# Autodesk Inventor assembly: ArmAssembly
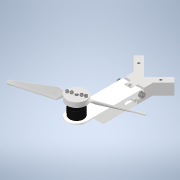
[picture p0: Inventor's stored thumbnail of the model, 180x180]
Saved by Autodesk Inventor 2021 (Build 250183000, 183)
## iProperties
Created: 2020-11-19
Part Number: ArmAssembly
Document SubType Name: Assembly
Designer: Pysion
Author: Pysion
## Documents named in this file (10)
- C:\Users\vineeth\Desktop\GrabCAD\Group 32 Assembly\ArmAssembly.iam
- C:\Users\vineeth\Desktop\GrabCAD\Group 32 Assembly\PropellerAssembly.iam
- C:\Users\vineeth\Desktop\GrabCAD\Group 32 Assembly\Motor.ipt
- C:\Users\vineeth\Desktop\GrabCAD\Group 32 Assembly\l_bracket.ipt
- C:\Users\vineeth\Desktop\GrabCAD\Group 32 Assembly\Motor Full Arm.ipt
- C:\Users\vineeth\Desktop\GrabCAD\Group 32 Assembly\slider.ipt
- C:\Users\vineeth\Desktop\GrabCAD\Group 32 Assembly\Compress Spring11.ipt
- C:\Users\vineeth\Desktop\GrabCAD\Group 32 Assembly\Pin GB 878-86 6 x 20.ipt
- C:\Users\vineeth\Desktop\GrabCAD\Group 32 Assembly\ContentCenter\en-US\AS 1420\AS 1420 - 1973 - M6 x 16.ipt
- C:\Users\vineeth\Documents\Inventor\Content Center Files\R2021\en-US\AS 1420\AS 1420 - 1973 - M4 x 10.ipt
## Components (14 placed, 9 different names)
1. PropellerAssembly:1 [sub-assembly] — Insert:1
2. Motor:1 — Mate:4, Mate:5, Mate:6, Insert:1
3. l_bracket:1 — Angle:1, Mate:8, Mate:21, Angle:3
4. Motor Full Arm:1 — Angle:1, Mate:4, Mate:5, Mate:6, Mate:8, Mate:17, Mate:18, Mate:19, Mate:20, Mate:21, Mate:22, Mate:23, Mate:24, Mate:25, Insert:2, Insert:3, Insert:4, Insert:5, Angle:7, Mate:26, Mate:29, Angle:8, Mate:30, Angle:9, Angle:10
5. slider:1 — Mate:26, Mate:27, Flush:1, Mate:29, Angle:8, Mate:30
6. Compress Spring1:1 — Mate:17, Mate:19, Angle:10
7. Screw GB/T 878-2007 6x20:1 — Mate:27, Flush:1
8. Compress Spring1:2 — Mate:18, Mate:20, Angle:9
9. AS 1420 - Metric M6 x 16:1 — Mate:22, Mate:23, Angle:2, Angle:3
10. AS 1420 - Metric M6 x 16:2 — Mate:24, Mate:25, Angle:2
11. AS 1420 - Metric M4 x 10:3 — Insert:5, Angle:6, Angle:7
12. AS 1420 - Metric M4 x 10:2 — Insert:4, Angle:5, Angle:6
13. AS 1420 - Metric M4 x 10:1 — Insert:3, Angle:4, Angle:5
14. AS 1420 - Metric M4 x 10:4 — Insert:2, Angle:4
## Relationships (33: Mate 17, Angle 10, Insert 5, Flush 1)
- Angle:1 (0 deg): l_bracket:1 ↔ Motor Full Arm:1
- Mate:4: Motor:1 ↔ Motor Full Arm:1
- Mate:5: Motor:1 ↔ Motor Full Arm:1
- Mate:6: Motor:1 ↔ Motor Full Arm:1
- Insert:1: PropellerAssembly:1 ↔ Motor:1
- Mate:8: l_bracket:1 ↔ Motor Full Arm:1
- Mate:17: Motor Full Arm:1 ↔ Compress Spring1:1
- Mate:18: Motor Full Arm:1 ↔ Compress Spring1:2
- Mate:19: Motor Full Arm:1 ↔ Compress Spring1:1
- Mate:20: Motor Full Arm:1 ↔ Compress Spring1:2
- Mate:21: l_bracket:1 ↔ Motor Full Arm:1
- Mate:22: Motor Full Arm:1 ↔ AS 1420 - Metric M6 x 16:1
- Mate:23: Motor Full Arm:1 ↔ AS 1420 - Metric M6 x 16:1
- Mate:24: Motor Full Arm:1 ↔ AS 1420 - Metric M6 x 16:2
- Mate:25: Motor Full Arm:1 ↔ AS 1420 - Metric M6 x 16:2
- Angle:2 (0 deg): AS 1420 - Metric M6 x 16:1 ↔ AS 1420 - Metric M6 x 16:2
- Angle:3 (0 deg): l_bracket:1 ↔ AS 1420 - Metric M6 x 16:1
- Insert:2: Motor Full Arm:1 ↔ AS 1420 - Metric M4 x 10:4
- Insert:3: Motor Full Arm:1 ↔ AS 1420 - Metric M4 x 10:1
- Insert:4: Motor Full Arm:1 ↔ AS 1420 - Metric M4 x 10:2
- Insert:5: Motor Full Arm:1 ↔ AS 1420 - Metric M4 x 10:3
- Angle:4 (0 deg): AS 1420 - Metric M4 x 10:1 ↔ AS 1420 - Metric M4 x 10:4
- Angle:5 (0 deg): AS 1420 - Metric M4 x 10:2 ↔ AS 1420 - Metric M4 x 10:1
- Angle:6 (0 deg): AS 1420 - Metric M4 x 10:3 ↔ AS 1420 - Metric M4 x 10:2
- Angle:7 (0 deg): Motor Full Arm:1 ↔ AS 1420 - Metric M4 x 10:3
- Mate:26: Motor Full Arm:1 ↔ slider:1
- Mate:27: slider:1 ↔ Screw GB/T 878-2007 6x20:1
- Flush:1: slider:1 ↔ Screw GB/T 878-2007 6x20:1
- Mate:29: Motor Full Arm:1 ↔ slider:1
- Angle:8 (0 deg): Motor Full Arm:1 ↔ slider:1
- Mate:30 (3 mm): Motor Full Arm:1 ↔ slider:1
- Angle:9 (0 deg): Motor Full Arm:1 ↔ Compress Spring1:2
- Angle:10 (0 deg): Motor Full Arm:1 ↔ Compress Spring1:1
